# Autodesk Inventor assembly: WCD V2
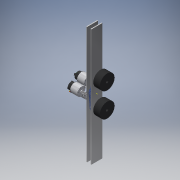
[picture p0: Inventor's stored thumbnail of the model, 180x180]
Saved by Autodesk Inventor 2019.4 (Build 234330000, 330)
## iProperties
Created: 2019-12-07
Part Number: WCD V2
Document SubType Name: Assembly
Designer: admin
Author: admin
## Documents named in this file (9)
- C:\Users\admin\Desktop\FRC 2020 Engineering\GitHub\7738-CAD-prep\WCD\WCD V2.iam
- C:\Users\admin\Desktop\FRC 2020 Engineering\GitHub\7738-CAD-prep\Swerve Module\Falcon_500_Powered_by_Talon_FX_217-6515.iam
- C:\Users\admin\Desktop\FRC 2020 Engineering\GitHub\7738-CAD-prep\WCD\50t_Aluminum_Spur_Gear_20_DP_1_2_Hex_Bore_217-3572.ipt
- C:\Users\admin\Desktop\FRC 2020 Engineering\GitHub\7738-CAD-prep\WCD\10T_Steel_Spur_Gear_20_DP_12T_Center_Distance_Falcon_Motor_217-6917.ipt
- C:\Users\admin\Desktop\FRC 2020 Engineering\GitHub\7738-CAD-prep\WCD\Wheel.ipt
- C:\Users\admin\Desktop\FRC 2020 Engineering\GitHub\7738-CAD-prep\WCD\WCD V2\Design Accelerator\Chain Drive1.iam
- C:\Users\admin\Desktop\FRC 2020 Engineering\GitHub\7738-CAD-prep\WCD\WCD V2\Design Accelerator\Chain Drive2.iam
- C:\Users\admin\Desktop\FRC 2020 Engineering\GitHub\7738-CAD-prep\WCD\Inner Plate.ipt
- C:\Users\admin\Desktop\FRC 2020 Engineering\GitHub\7738-CAD-prep\WCD\Outer Plate.ipt
## Components (13 placed, 7 different names)
1. Wheel:1 — Flush:7, Mate:12, Mate:15, Mate:16, Mate:17, Mate:21
2. Wheel:2 — Flush:7, Mate:14
3. Chain Drive:1 [sub-assembly] — Mate:14, Mate:19
4. Chain Drive:2 [sub-assembly] — Mate:15, Mate:16
5. Inner Plate:1 — Mate:17, Angle:1, Mate:21, Mate:22, Flush:10, Flush:11
6. Outer Plate:1 — Mate:22, Flush:10, Flush:11
7. Falcon_500_Powered_by_Talon_FX_217-6515:1 [sub-assembly] — Mate:2, Flush:4, Mate:8, Mate:11
8. Falcon_500_Powered_by_Talon_FX_217-6515:2 [sub-assembly] — Mate:1, Flush:3, Mate:7, Mate:8, Flush:9
9. Falcon_500_Powered_by_Talon_FX_217-6515:3 [sub-assembly] — Mate:3, Flush:2, Mate:7, Mate:10
10. 50t_Aluminum_Spur_Gear_20_DP_1_2_Hex_Bore_217-3572:1 — Mate:4, Mate:5, Mate:6, Flush:1, Flush:5, Flush:6, Mate:19
11. 10T_Steel_Spur_Gear_20_DP_12T_Center_Distance_Falcon_Motor_217-6917:1 — Mate:1, Mate:5, Flush:3, Flush:6
12. 10T_Steel_Spur_Gear_20_DP_12T_Center_Distance_Falcon_Motor_217-6917:2 — Mate:2, Mate:4, Flush:4, Flush:5
13. 10T_Steel_Spur_Gear_20_DP_12T_Center_Distance_Falcon_Motor_217-6917:3 — Mate:3, Mate:6, Flush:1, Flush:2
## Relationships (30: Mate 18, Flush 11, Angle 1)
- Mate:1: Falcon_500_Powered_by_Talon_FX_217-6515:2 ↔ 10T_Steel_Spur_Gear_20_DP_12T_Center_Distance_Falcon_Motor_217-6917:1
- Mate:2: Falcon_500_Powered_by_Talon_FX_217-6515:1 ↔ 10T_Steel_Spur_Gear_20_DP_12T_Center_Distance_Falcon_Motor_217-6917:2
- Mate:3: Falcon_500_Powered_by_Talon_FX_217-6515:3 ↔ 10T_Steel_Spur_Gear_20_DP_12T_Center_Distance_Falcon_Motor_217-6917:3
- Mate:4 (39.37 mm): 50t_Aluminum_Spur_Gear_20_DP_1_2_Hex_Bore_217-3572:1 ↔ 10T_Steel_Spur_Gear_20_DP_12T_Center_Distance_Falcon_Motor_217-6917:2
- Mate:5 (39.37 mm): 50t_Aluminum_Spur_Gear_20_DP_1_2_Hex_Bore_217-3572:1 ↔ 10T_Steel_Spur_Gear_20_DP_12T_Center_Distance_Falcon_Motor_217-6917:1
- Mate:6 (39.37 mm): 50t_Aluminum_Spur_Gear_20_DP_1_2_Hex_Bore_217-3572:1 ↔ 10T_Steel_Spur_Gear_20_DP_12T_Center_Distance_Falcon_Motor_217-6917:3
- Flush:1 (-5 mm): 50t_Aluminum_Spur_Gear_20_DP_1_2_Hex_Bore_217-3572:1 ↔ 10T_Steel_Spur_Gear_20_DP_12T_Center_Distance_Falcon_Motor_217-6917:3
- Flush:2 (-8 mm): Falcon_500_Powered_by_Talon_FX_217-6515:3 ↔ 10T_Steel_Spur_Gear_20_DP_12T_Center_Distance_Falcon_Motor_217-6917:3
- Flush:3 (-8 mm): Falcon_500_Powered_by_Talon_FX_217-6515:2 ↔ 10T_Steel_Spur_Gear_20_DP_12T_Center_Distance_Falcon_Motor_217-6917:1
- Flush:4 (8 mm): Falcon_500_Powered_by_Talon_FX_217-6515:1 ↔ 10T_Steel_Spur_Gear_20_DP_12T_Center_Distance_Falcon_Motor_217-6917:2
- Flush:5 (-5 mm): 50t_Aluminum_Spur_Gear_20_DP_1_2_Hex_Bore_217-3572:1 ↔ 10T_Steel_Spur_Gear_20_DP_12T_Center_Distance_Falcon_Motor_217-6917:2
- Flush:6 (-5 mm): 50t_Aluminum_Spur_Gear_20_DP_1_2_Hex_Bore_217-3572:1 ↔ 10T_Steel_Spur_Gear_20_DP_12T_Center_Distance_Falcon_Motor_217-6917:1
- Mate:7 (61 mm): Falcon_500_Powered_by_Talon_FX_217-6515:2 ↔ Falcon_500_Powered_by_Talon_FX_217-6515:3
- Mate:8 (61 mm): Falcon_500_Powered_by_Talon_FX_217-6515:1 ↔ Falcon_500_Powered_by_Talon_FX_217-6515:2
- Flush:7: Wheel:1 ↔ Wheel:2
- Mate:10: Falcon_500_Powered_by_Talon_FX_217-6515:3
- Mate:11: Falcon_500_Powered_by_Talon_FX_217-6515:1
- Flush:8 (20 mm)
- Mate:12: Wheel:1
- Flush:9: Falcon_500_Powered_by_Talon_FX_217-6515:2
- Mate:14: Wheel:2 ↔ Chain Drive:1
- Mate:15 (16 mm): Wheel:1 ↔ Chain Drive:2
- Mate:16: Wheel:1 ↔ Chain Drive:2
- Mate:17 (3 mm): Wheel:1 ↔ Inner Plate:1
- Mate:19: Chain Drive:1 ↔ 50t_Aluminum_Spur_Gear_20_DP_1_2_Hex_Bore_217-3572:1
- Angle:1 (0 deg): Inner Plate:1
- Mate:21: Wheel:1 ↔ Inner Plate:1
- Mate:22 (23 mm): Inner Plate:1 ↔ Outer Plate:1
- Flush:10: Inner Plate:1 ↔ Outer Plate:1
- Flush:11: Inner Plate:1 ↔ Outer Plate:1
